# Autodesk Inventor assembly: Omnidirectional_Robot
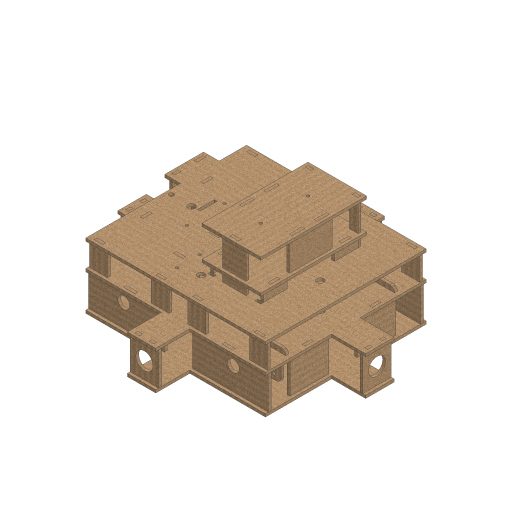
[picture p0: Inventor's stored thumbnail of the model, 512x512]
Saved by Autodesk Inventor 2024 (Build 280153000, 153)
## iProperties
Created: 2023-11-26
Part Number: Omnidirectional_Robot
Document SubType Name: Assembly
Designer: marco
Author: marco
## Documents named in this file (18)
- C:\Users\marco\OneDrive\Documents\Omnidirectional_Robot\Omnidirectional_Robot.iam
- C:\Users\marco\OneDrive\Documents\Omnidirectional_Robot\Base2.ipt
- C:\Users\marco\OneDrive\Documents\Omnidirectional_Robot\Motor_Support.ipt
- C:\Users\marco\OneDrive\Documents\Omnidirectional_Robot\Wheel_Support.ipt
- C:\Users\marco\OneDrive\Documents\Omnidirectional_Robot\Wall_Base1.ipt
- C:\Users\marco\OneDrive\Documents\Omnidirectional_Robot\Sensor_Support.ipt
- C:\Users\marco\OneDrive\Documents\Omnidirectional_Robot\Battery_Wall1.ipt
- C:\Users\marco\OneDrive\Documents\Omnidirectional_Robot\Battery_Wall2.ipt
- C:\Users\marco\OneDrive\Documents\Omnidirectional_Robot\Base1.ipt
- C:\Users\marco\OneDrive\Documents\Omnidirectional_Robot\Base3.ipt
- C:\Users\marco\OneDrive\Documents\Omnidirectional_Robot\Switch_Support.ipt
- C:\Users\marco\OneDrive\Documents\Omnidirectional_Robot\Wall_Base2.ipt
- C:\Users\marco\OneDrive\Documents\Omnidirectional_Robot\Case_Support.ipt
- C:\Users\marco\OneDrive\Documents\Omnidirectional_Robot\Case_Base1.ipt
- C:\Users\marco\OneDrive\Documents\Omnidirectional_Robot\Case_Wall3.ipt
- C:\Users\marco\OneDrive\Documents\Omnidirectional_Robot\Case_Wall2.ipt
- C:\Users\marco\OneDrive\Documents\Omnidirectional_Robot\Case_Wall1.ipt
- C:\Users\marco\OneDrive\Documents\Omnidirectional_Robot\Case_Base2.ipt
## Components (47 placed, 17 different names)
1. Base2:1 — Corredera:1, Corredera:2, Corredera:3, Corredera:4, Rígido:1, Rígido:2, Rígido:3, Rígido:4, Rígido:5, Rígido:6, Rígido:7, Rígido:8, Rígido:9, Rígido:10, Rígido:11, Rígido:12, Rígido:13, Rígido:14, Rígido:15, Rígido:16, Rígido:17, Rígido:18, Rígido:19, Rígido:20, Rígido:23, Rígido:24, Rígido:25, Rígido:26, Rígido:27, Rígido:28, Rígido:29, Rígido:30, Rígido:36
2. Motor_Support:1 — Corredera:4
3. Motor_Support:2 — Corredera:3
4. Motor_Support:3 — Corredera:1
5. Motor_Support:4 — Corredera:2
6. Wheel_Support:1 — Rígido:7
7. Wheel_Support:2 — Rígido:5
8. Wheel_Support:3 — Rígido:6
9. Wheel_Support:4 — Rígido:8
10. Wall_Base1:1 — Rígido:3
11. Wall_Base1:2 — Rígido:1
12. Wall_Base1:3 — Rígido:2
13. Wall_Base1:4 — Rígido:4
14. Sensor_Support:1 — Rígido:10
15. Sensor_Support:2 — Rígido:9
16. Sensor_Support:3 — Rígido:11
17. Sensor_Support:4 — Rígido:12, Rígido:21
18. Battery_Wall1:1 — Rígido:17
19. Battery_Wall1:2 — Rígido:19
20. Battery_Wall1:3 — Rígido:18
21. Battery_Wall1:4 — Rígido:20
22. Battery_Wall2:1 — Rígido:13
23. Battery_Wall2:2 — Rígido:15
24. Battery_Wall2:3 — Rígido:14
25. Battery_Wall2:4 — Rígido:16
26. Base1:1 — Rígido:21
27. Base3:1 — Rígido:32, Rígido:33, Rígido:34, Rígido:35, Rígido:37, Rígido:42, Rígido:43, Rígido:44
28. Wall_Base2:1 — Rígido:27
29. Wall_Base2:2 — Rígido:23
30. Wall_Base2:3 — Rígido:24
31. Wall_Base2:4 — Rígido:25
32. Wall_Base2:5 — Rígido:26
33. Wall_Base2:6 — Rígido:30
34. Wall_Base2:7 — Rígido:28
35. Wall_Base2:8 — Rígido:29
36. Case_Support:1 — Rígido:35, Rígido:41
37. Case_Support:2 — Rígido:33, Rígido:39
38. Case_Support:3 — Rígido:34, Rígido:40
39. Case_Support:4 — Rígido:32, Rígido:38
40. Switch_Support:2 — Rígido:36, Rígido:37
41. Case_Base1:1 — Rígido:38, Rígido:39, Rígido:40, Rígido:41, Rígido:45, Rígido:46
42. Case_Wall3:1 — Rígido:43, Rígido:47
43. Case_Wall3:2 — Rígido:44, Rígido:48
44. Case_Wall2:1 — Rígido:46, Rígido:50
45. Case_Wall2:2 — Rígido:45, Rígido:49
46. Case_Wall1:1 — Rígido:42, Rígido:51
47. Case_Base2:1 — Rígido:47, Rígido:48, Rígido:49, Rígido:50, Rígido:51
## Relationships (53: WeldJoint 49, TranslationJoint 4)
- Corredera:1 [TranslationJoint]: Base2:1 ↔ Motor_Support:3
- Corredera:2 [TranslationJoint]: Base2:1 ↔ Motor_Support:4
- Corredera:3 [TranslationJoint]: Base2:1 ↔ Motor_Support:2
- Corredera:4 [TranslationJoint]: Base2:1 ↔ Motor_Support:1
- Rígido:1 [WeldJoint]: Base2:1 ↔ Wall_Base1:2
- Rígido:2 [WeldJoint]: Base2:1 ↔ Wall_Base1:3
- Rígido:3 [WeldJoint]: Base2:1 ↔ Wall_Base1:1
- Rígido:4 [WeldJoint]: Base2:1 ↔ Wall_Base1:4
- Rígido:5 [WeldJoint]: Base2:1 ↔ Wheel_Support:2
- Rígido:6 [WeldJoint]: Base2:1 ↔ Wheel_Support:3
- Rígido:7 [WeldJoint]: Base2:1 ↔ Wheel_Support:1
- Rígido:8 [WeldJoint]: Base2:1 ↔ Wheel_Support:4
- Rígido:9 [WeldJoint]: Base2:1 ↔ Sensor_Support:2
- Rígido:10 [WeldJoint]: Base2:1 ↔ Sensor_Support:1
- Rígido:11 [WeldJoint]: Base2:1 ↔ Sensor_Support:3
- Rígido:12 [WeldJoint]: Base2:1 ↔ Sensor_Support:4
- Rígido:13 [WeldJoint]: Base2:1 ↔ Battery_Wall2:1
- Rígido:14 [WeldJoint]: Base2:1 ↔ Battery_Wall2:3
- Rígido:15 [WeldJoint]: Base2:1 ↔ Battery_Wall2:2
- Rígido:16 [WeldJoint]: Base2:1 ↔ Battery_Wall2:4
- Rígido:17 [WeldJoint]: Base2:1 ↔ Battery_Wall1:1
- Rígido:18 [WeldJoint]: Base2:1 ↔ Battery_Wall1:3
- Rígido:19 [WeldJoint]: Base2:1 ↔ Battery_Wall1:2
- Rígido:20 [WeldJoint]: Base2:1 ↔ Battery_Wall1:4
- Rígido:21 [WeldJoint]: Sensor_Support:4 ↔ Base1:1
- Rígido:23 [WeldJoint]: Base2:1 ↔ Wall_Base2:2
- Rígido:24 [WeldJoint]: Base2:1 ↔ Wall_Base2:3
- Rígido:25 [WeldJoint]: Base2:1 ↔ Wall_Base2:4
- Rígido:26 [WeldJoint]: Base2:1 ↔ Wall_Base2:5
- Rígido:27 [WeldJoint]: Base2:1 ↔ Wall_Base2:1
- Rígido:28 [WeldJoint]: Base2:1 ↔ Wall_Base2:7
- Rígido:29 [WeldJoint]: Base2:1 ↔ Wall_Base2:8
- Rígido:30 [WeldJoint]: Base2:1 ↔ Wall_Base2:6
- Rígido:32 [WeldJoint]: Base3:1 ↔ Case_Support:4
- Rígido:33 [WeldJoint]: Base3:1 ↔ Case_Support:2
- Rígido:34 [WeldJoint]: Base3:1 ↔ Case_Support:3
- Rígido:35 [WeldJoint]: Base3:1 ↔ Case_Support:1
- Rígido:36 [WeldJoint]: Base2:1 ↔ Switch_Support:2
- Rígido:37 [WeldJoint]: Base3:1 ↔ Switch_Support:2
- Rígido:38 [WeldJoint]: Case_Support:4 ↔ Case_Base1:1
- Rígido:39 [WeldJoint]: Case_Support:2 ↔ Case_Base1:1
- Rígido:40 [WeldJoint]: Case_Support:3 ↔ Case_Base1:1
- Rígido:41 [WeldJoint]: Case_Support:1 ↔ Case_Base1:1
- Rígido:42 [WeldJoint]: Base3:1 ↔ Case_Wall1:1
- Rígido:43 [WeldJoint]: Base3:1 ↔ Case_Wall3:1
- Rígido:44 [WeldJoint]: Base3:1 ↔ Case_Wall3:2
- Rígido:45 [WeldJoint]: Case_Base1:1 ↔ Case_Wall2:2
- Rígido:46 [WeldJoint]: Case_Base1:1 ↔ Case_Wall2:1
- Rígido:47 [WeldJoint]: Case_Wall3:1 ↔ Case_Base2:1
- Rígido:48 [WeldJoint]: Case_Wall3:2 ↔ Case_Base2:1
- Rígido:49 [WeldJoint]: Case_Wall2:2 ↔ Case_Base2:1
- Rígido:50 [WeldJoint]: Case_Wall2:1 ↔ Case_Base2:1
- Rígido:51 [WeldJoint]: Case_Wall1:1 ↔ Case_Base2:1
